# Autodesk Inventor assembly: Vial Carousel
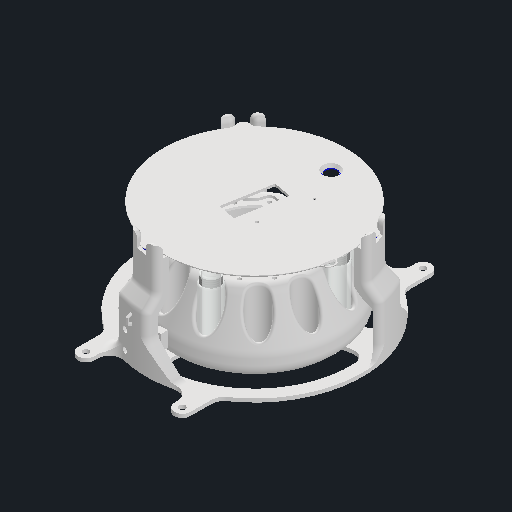
[picture p0: Inventor's stored thumbnail of the model, 512x512]
Saved by Autodesk Inventor 2026 (Build 300175000, 175)
## iProperties
Created: 2025-02-21
Part Number: Vial Carousel
Document SubType Name: Assembly
Designer: jerem
Author: jerem
## Documents named in this file (8)
- C:\Users\jerem\Documents\GitHub\Perovskite-Automated-Synthesis-System\CAD\vial carousel\Vial Carousel.iam
- C:\Users\jerem\Documents\GitHub\Perovskite-Automated-Synthesis-System\CAD\Non 3D Printed Parts\Motors and Servos\NEMA17 Stepper Motor - 26 mm.ipt
- C:\Users\jerem\Documents\GitHub\Perovskite-Automated-Synthesis-System\CAD\vial carousel\Vial Holder.ipt
- C:\Users\jerem\Documents\GitHub\Perovskite-Automated-Synthesis-System\CAD\Non 3D Printed Parts\Vial.ipt
- C:\Users\jerem\Documents\GitHub\Perovskite-Automated-Synthesis-System\CAD\vial carousel\Motor Mount.ipt
- C:\Users\jerem\Documents\GitHub\Perovskite-Automated-Synthesis-System\CAD\vial carousel\Shaft Collar.ipt
- C:\Users\jerem\Documents\GitHub\Perovskite-Automated-Synthesis-System\CAD\vial carousel\Vial Cover.ipt
- C:\Users\jerem\Documents\GitHub\Perovskite-Automated-Synthesis-System\CAD\Non 3D Printed Parts\Limit Switch.ipt
## Components (12 placed, 7 different names)
1. NEMA17 Stepper Motor - 26 mm:1 — Mate:7, Mate:8, Mate:9, Mate:11, Mate:19, Mate:22
2. Vial Holder:1 — Mate:1, Mate:2, Mate:3, Mate:4, Mate:5, Mate:6, Mate:19, Mate:20, Mate:23, Mate:24, Mate:25, Mate:26, Mate:56, Mate:57, Mate:58, Mate:59
3. Vial:1 — Mate:4, Mate:5
4. Vial:2 — Mate:3, Mate:6
5. Vial:3 — Mate:1, Mate:2
6. Motor Mount:1 — Mate:7, Mate:8, Mate:9, Mate:28, Mate:29, Mate:30, Mate:66
7. Shaft Collar:1 — Mate:11, Mate:20, Mate:22, Mate:23
8. Vial Cover:1 — Mate:24, Mate:66
9. Vial:4 — Mate:25, Mate:26
10. Limit Switch:1 — Mate:28, Mate:29, Mate:30
11. Vial:5 — Mate:56, Mate:57
12. Vial:6 — Mate:58, Mate:59
## Relationships (25: Mate 25)
- Mate:1: Vial Holder:1 ↔ Vial:3
- Mate:2: Vial Holder:1 ↔ Vial:3
- Mate:3: Vial Holder:1 ↔ Vial:2
- Mate:4: Vial Holder:1 ↔ Vial:1
- Mate:5: Vial Holder:1 ↔ Vial:1
- Mate:6: Vial Holder:1 ↔ Vial:2
- Mate:7: NEMA17 Stepper Motor - 26 mm:1 ↔ Motor Mount:1
- Mate:8: NEMA17 Stepper Motor - 26 mm:1 ↔ Motor Mount:1
- Mate:9: NEMA17 Stepper Motor - 26 mm:1 ↔ Motor Mount:1
- Mate:11: NEMA17 Stepper Motor - 26 mm:1 ↔ Shaft Collar:1
- Mate:19: NEMA17 Stepper Motor - 26 mm:1 ↔ Vial Holder:1
- Mate:20: Vial Holder:1 ↔ Shaft Collar:1
- Mate:22: NEMA17 Stepper Motor - 26 mm:1 ↔ Shaft Collar:1
- Mate:23: Vial Holder:1 ↔ Shaft Collar:1
- Mate:24: Vial Holder:1 ↔ Vial Cover:1
- Mate:25: Vial Holder:1 ↔ Vial:4
- Mate:26: Vial Holder:1 ↔ Vial:4
- Mate:28: Motor Mount:1 ↔ Limit Switch:1
- Mate:29: Motor Mount:1 ↔ Limit Switch:1
- Mate:30: Motor Mount:1 ↔ Limit Switch:1
- Mate:56: Vial Holder:1 ↔ Vial:5
- Mate:57: Vial Holder:1 ↔ Vial:5
- Mate:58: Vial Holder:1 ↔ Vial:6
- Mate:59: Vial Holder:1 ↔ Vial:6
- Mate:66: Motor Mount:1 ↔ Vial Cover:1
